# Autodesk Inventor assembly: axis5_6
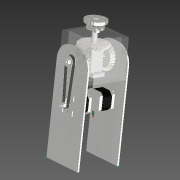
[picture p0: Inventor's stored thumbnail of the model, 180x180]
Saved by Autodesk Inventor 2020 (Build 240168000, 168)
## iProperties
Created: 2020-05-15
Part Number: axis5_6
Document SubType Name: Assembly
Designer: stefa
Author: stefa
## Documents named in this file (15)
- D:\github_gedeeld\BeerMinder\3D-model\axis5_6\axis5_6.iam
- D:\github_gedeeld\BeerMinder\3D-model\pulleys\tandriem32Tnaar16T_lengte240.ipt
- D:\github_gedeeld\BeerMinder\3D-model\pulleys\GT2 Timing Pulley 36T - 8mm as.ipt
- D:\github_gedeeld\BeerMinder\3D-model\stepper motors\42BYG Stepper Motor.ipt
- D:\github_gedeeld\BeerMinder\3D-model\pulleys\GT2 Pulley 16T - 5mm as.ipt
- D:\github_gedeeld\BeerMinder\3D-model\axis5_6\axis5_6\Design Accelerator\Bevel Gears1.iam
- D:\github_gedeeld\BeerMinder\3D-model\axis5_6\endeffector mount part.ipt
- D:\github_gedeeld\BeerMinder\3D-model\axis5_6\bovenarm - links.ipt
- D:\github_gedeeld\BeerMinder\3D-model\axis5_6\as naar endeffector.ipt
- D:\github_gedeeld\BeerMinder\3D-model\axis5_6\axis5_6\Design Accelerator\Bevel Gear11.ipt
- D:\github_gedeeld\BeerMinder\3D-model\bearings\bloklager.ipt
- D:\github_gedeeld\BeerMinder\3D-model\axis5_6\3 dubbele lagerblok assemble.iam
- D:\github_gedeeld\BeerMinder\3D-model\axis5_6\draaideel voor endeffector.ipt
- D:\github_gedeeld\BeerMinder\3D-model\bearings\Ball Bearing 608ZZ.ipt
- D:\github_gedeeld\BeerMinder\3D-model\axis5_6\as bevelgear.ipt
## Components (21 placed, 14 different names)
1. tandriem32Tnaar16T_lengte240:1 — Mate:57, Mate:58, Mate:106, Mate:107
2. tandriem32Tnaar16T_lengte240:2 — Mate:60, Mate:89, Mate:94, Mate:100
3. Bevel Gears:1 [sub-assembly] — Mate:28, Mate:38, Mate:39, Mate:68, Mate:72
4. 42BYG Stepper Motor:2 — Mate:96, Mate:108, Flush:12
5. endeffector mount part:1 — Mate:27, Flush:5, Mate:85
6. bovenarm - links:1 — Angle:3, Flush:6, Flush:7, Mate:96, Flush:12, Mate:109
7. as naar endeffector:1 — Mate:27, Mate:28, Mate:81, Flush:5
8. Bevel Gear1:1 — Mate:38, Mate:39, Mate:83
9. GT2 Timing Pulley 36T - 8mm as:6 — Mate:57, Mate:58, Mate:76
10. GT2 Timing Pulley 36T - 8mm as:7 — Mate:60, Mate:79, Mate:100, Flush:11
11. bovenarm - links:2 — Flush:6, Flush:7, Mate:84, Mate:99, Mate:102, Flush:10, Mate:103, Mate:104, Mate:105
12. 3 dubbele lagerblok assemble:1 [sub-assembly] — Mate:68, Mate:71, Mate:77, Mate:80, Mate:81, Mate:82
13. draaideel voor endeffector:1 — Mate:71, Flush:8, Mate:86, Mate:87, Flush:9
14. bloklager:1 — Mate:72, Mate:85
15. Ball Bearing 608ZZ:1 — Mate:75, Flush:8, Mate:86
16. Ball Bearing 608ZZ:2 — Mate:78, Mate:87, Flush:9
17. as bevelgear:1 — Mate:75, Mate:76, Mate:77
18. as bevelgear:2 — Mate:78, Mate:79, Mate:80, Mate:82, Mate:83, Mate:84, Flush:11
19. GT2 Pulley 16T - 5mm as:2 — Mate:89, Mate:94, Mate:101, Mate:102
20. GT2 Pulley 16T - 5mm as:3 — Mate:106, Mate:107, Mate:108, Mate:109
21. 42BYG Stepper Motor:3 — Mate:99, Mate:101, Flush:10
## Relationships (46: Mate 37, Flush 8, Angle 1)
- Mate:27: endeffector mount part:1 ↔ as naar endeffector:1
- Mate:28: Bevel Gears:1 ↔ as naar endeffector:1
- Angle:3 (0 deg): bovenarm - links:1
- Mate:38: Bevel Gears:1 ↔ Bevel Gear1:1
- Mate:39 (27.591 mm): Bevel Gears:1 ↔ Bevel Gear1:1
- Mate:57 (0.5 mm): tandriem32Tnaar16T_lengte240:1 ↔ GT2 Timing Pulley 36T - 8mm as:6
- Mate:58: tandriem32Tnaar16T_lengte240:1 ↔ GT2 Timing Pulley 36T - 8mm as:6
- Mate:60 (0.5 mm): tandriem32Tnaar16T_lengte240:2 ↔ GT2 Timing Pulley 36T - 8mm as:7
- Mate:68: Bevel Gears:1 ↔ 3 dubbele lagerblok assemble:1
- Mate:71: 3 dubbele lagerblok assemble:1 ↔ draaideel voor endeffector:1
- Mate:72: Bevel Gears:1 ↔ bloklager:1
- Mate:75: Ball Bearing 608ZZ:1 ↔ as bevelgear:1
- Mate:76: GT2 Timing Pulley 36T - 8mm as:6 ↔ as bevelgear:1
- Mate:77 (-9 mm): 3 dubbele lagerblok assemble:1 ↔ as bevelgear:1
- Mate:78: Ball Bearing 608ZZ:2 ↔ as bevelgear:2
- Mate:79: GT2 Timing Pulley 36T - 8mm as:7 ↔ as bevelgear:2
- Mate:80 (-8 mm): 3 dubbele lagerblok assemble:1 ↔ as bevelgear:2
- Mate:81 (-9 mm): as naar endeffector:1 ↔ 3 dubbele lagerblok assemble:1
- Flush:5: endeffector mount part:1 ↔ as naar endeffector:1
- Flush:6: bovenarm - links:1 ↔ bovenarm - links:2
- Flush:7: bovenarm - links:1 ↔ bovenarm - links:2
- Mate:82: 3 dubbele lagerblok assemble:1 ↔ as bevelgear:2
- Mate:83: Bevel Gear1:1 ↔ as bevelgear:2
- Mate:84: bovenarm - links:2 ↔ as bevelgear:2
- Mate:85 (2 mm): endeffector mount part:1 ↔ bloklager:1
- Flush:8: draaideel voor endeffector:1 ↔ Ball Bearing 608ZZ:1
- Mate:86: draaideel voor endeffector:1 ↔ Ball Bearing 608ZZ:1
- Mate:87: draaideel voor endeffector:1 ↔ Ball Bearing 608ZZ:2
- Flush:9: draaideel voor endeffector:1 ↔ Ball Bearing 608ZZ:2
- Mate:89 (0.5 mm): tandriem32Tnaar16T_lengte240:2 ↔ GT2 Pulley 16T - 5mm as:2
- Mate:94: tandriem32Tnaar16T_lengte240:2 ↔ GT2 Pulley 16T - 5mm as:2
- Mate:96: 42BYG Stepper Motor:2 ↔ bovenarm - links:1
- Mate:99: bovenarm - links:2 ↔ 42BYG Stepper Motor:3
- Mate:100: tandriem32Tnaar16T_lengte240:2 ↔ GT2 Timing Pulley 36T - 8mm as:7
- Mate:101: GT2 Pulley 16T - 5mm as:2 ↔ 42BYG Stepper Motor:3
- Mate:102 (2 mm): bovenarm - links:2 ↔ GT2 Pulley 16T - 5mm as:2
- Flush:10 (-6.55 mm): bovenarm - links:2 ↔ 42BYG Stepper Motor:3
- Mate:103: bovenarm - links:2
- Mate:104: bovenarm - links:2
- Mate:105: bovenarm - links:2
- Flush:11 (-2 mm): GT2 Timing Pulley 36T - 8mm as:7 ↔ as bevelgear:2
- Mate:106: tandriem32Tnaar16T_lengte240:1 ↔ GT2 Pulley 16T - 5mm as:3
- Mate:107 (0.5 mm): tandriem32Tnaar16T_lengte240:1 ↔ GT2 Pulley 16T - 5mm as:3
- Mate:108: 42BYG Stepper Motor:2 ↔ GT2 Pulley 16T - 5mm as:3
- Flush:12 (6.8 mm): 42BYG Stepper Motor:2 ↔ bovenarm - links:1
- Mate:109 (2 mm): bovenarm - links:1 ↔ GT2 Pulley 16T - 5mm as:3
